# Autodesk Inventor assembly: Servo Arm
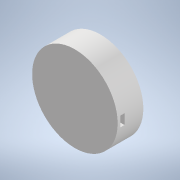
[picture p0: Inventor's stored thumbnail of the model, 180x180]
Saved by Autodesk Inventor 2020 (Build 240168000, 168)
## iProperties
Created: 2020-02-27
Part Number: Servo Arm
Document SubType Name: Assembly
Designer: othscs164
Author: othscs164
## Documents named in this file (3)
- C:\Users\othscs164\Desktop\ServoArm\Servo Arm.iam
- C:\Users\othscs164\Desktop\ServoArm\Rotator Platform.ipt
- C:\Users\othscs164\Downloads\MicroServo9g.iam
## Components (2 placed, 2 different names)
1. Rotator Platform:1 — Mate:1, Mate:2, Mate:3
2. MicroServo9g:1 [sub-assembly] — Mate:1, Mate:2, Mate:3
## Relationships (3: Mate 3)
- Mate:1: Rotator Platform:1 ↔ MicroServo9g:1
- Mate:2: Rotator Platform:1 ↔ MicroServo9g:1
- Mate:3: Rotator Platform:1 ↔ MicroServo9g:1
